# Autodesk Inventor assembly: Z Drive Assembly
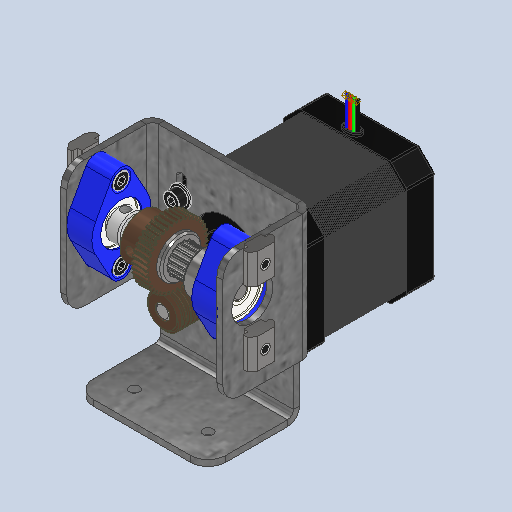
[picture p0: Inventor's stored thumbnail of the model, 512x512]
Saved by Autodesk Inventor 2022 (Build 260153000, 153)
## iProperties
Created: 2022-02-13
Part Number: Z Drive Assembly
Document SubType Name: Assembly
Designer: nicol
Author: nicol
## Documents named in this file (14)
- Y:\Projects\Bibble0\SubAsm\Z Drive Assembly.iam
- Y:\Projects\Bibble0\Sheet Metal\Z Drive Mount.ipt
- Y:\Projects\Bibble0\3D printed\Z Axis\Z Drive Bearing Holder.ipt
- Y:\Projects\Bibble0\Bearings\625 Bearing.ipt
- Y:\Projects\Bibble0\Hardware\5 x 50mm Shaft.ipt
- Y:\Projects\Bibble0\Hardware\GT2 Pulley 16T.ipt
- Y:\Projects\Bibble0\Hardware\METAL WORM GEAR_57545K624 v5.ipt
- Y:\Projects\Bibble0\Hardware\PLASTIC WORM GEAR_4037N115 v3.ipt
- Y:\Projects\Bibble0\Electronics\NEMA 17.ipt
- Y:\Projects\Bibble0\Hardware\M3 x 12 mm  SHCS.ipt
- Y:\Projects\Bibble0\Hardware\M3 T-Slot Nut.ipt
- Y:\Projects\Bibble0\Hardware\M3 x 6 mm SHCS.ipt
- Y:\Projects\Bibble0\Hardware\M3 Washer.ipt
- Y:\Projects\Bibble0\Hardware\5mm Collar.ipt
## Components (27 placed, 13 different names)
1. Z Drive Mount:1 — Insert:4, Insert:5, Insert:6, Mate:5, Insert:8, Insert:9, Insert:14, Insert:15, Insert:16, Insert:17, Angle:2, Angle:4, Insert:19, Insert:23, Insert:24, Insert:25
2. Z Drive Bearing Holder:1 — Insert:4, Insert:5, Insert:12, Insert:13
3. Z Drive Bearing Holder:2 — Insert:6, Insert:10, Insert:11
4. 625 Bearing:1 — Mate:4, Mate:6
5. 625 Bearing:2
6. 5 x 50mm Shaft:1 — Mate:4, Mate:7
7. GT2 Pulley 16T:1
8. METAL WORM GEAR_57545K624 v5:1 — Insert:7
9. PLASTIC WORM GEAR_4037N115 v3:1
10. NEMA 17:1 — Mate:5, Insert:7, Insert:8, Insert:9
11. M3 x 12 mm  SHCS:1 — Insert:10
12. M3 x 12 mm  SHCS:2 — Insert:12
13. M3 x 12 mm  SHCS:3 — Insert:11
14. M3 x 12 mm  SHCS:4 — Insert:13
15. M3 T-Slot Nut:1 — Insert:15, Angle:3, Angle:4
16. M3 T-Slot Nut:2 — Insert:17, Angle:1
17. M3 T-Slot Nut:3 — Insert:16, Angle:1, Angle:2
18. M3 T-Slot Nut:4 — Insert:14, Angle:3
19. M3 x 6 mm SHCS:1 — Insert:18
20. M3 Washer:1 — Insert:18, Insert:19
21. M3 x 6 mm SHCS:2
22. M3 Washer:2 — Insert:23
23. M3 x 6 mm SHCS:3
24. M3 Washer:3 — Insert:24
25. M3 x 6 mm SHCS:4
26. M3 Washer:4 — Insert:25
27. 5mm Collar:1 — Mate:6, Mate:7
## Relationships (37: Insert 25, Mate 7, Angle 4, Flush 1)
- [Insert]: Z Drive Bearing Holder:2 ↔ 625 Bearing:1
- [Insert]: Z Drive Bearing Holder:1 ↔ 625 Bearing:2
- [Mate]: 625 Bearing:2 ↔ 5 x 50mm Shaft:1
- [Flush]: 625 Bearing:2 ↔ 5 x 50mm Shaft:1
- [Insert]: GT2 Pulley 16T:1 ↔ PLASTIC WORM GEAR_4037N115 v3:1
- [Mate] (15 mm): Z Drive Bearing Holder:1 ↔ PLASTIC WORM GEAR_4037N115 v3:1
- [Mate]: 5 x 50mm Shaft:1 ↔ PLASTIC WORM GEAR_4037N115 v3:1
- Mate:4: 625 Bearing:1 ↔ 5 x 50mm Shaft:1
- Insert:4: Z Drive Mount:1 ↔ Z Drive Bearing Holder:1
- Insert:5: Z Drive Mount:1 ↔ Z Drive Bearing Holder:1
- Insert:6: Z Drive Mount:1 ↔ Z Drive Bearing Holder:2
- Mate:5: Z Drive Mount:1 ↔ NEMA 17:1
- Insert:7: METAL WORM GEAR_57545K624 v5:1 ↔ NEMA 17:1
- Insert:8: Z Drive Mount:1 ↔ NEMA 17:1
- Insert:9: Z Drive Mount:1 ↔ NEMA 17:1
- Insert:10: Z Drive Bearing Holder:2 ↔ M3 x 12 mm  SHCS:1
- Insert:11: Z Drive Bearing Holder:2 ↔ M3 x 12 mm  SHCS:3
- Insert:12: Z Drive Bearing Holder:1 ↔ M3 x 12 mm  SHCS:2
- Insert:13: Z Drive Bearing Holder:1 ↔ M3 x 12 mm  SHCS:4
- Insert:14: Z Drive Mount:1 ↔ M3 T-Slot Nut:4
- Insert:15: Z Drive Mount:1 ↔ M3 T-Slot Nut:1
- Insert:16: Z Drive Mount:1 ↔ M3 T-Slot Nut:3
- Insert:17: Z Drive Mount:1 ↔ M3 T-Slot Nut:2
- Angle:1 (0 deg): M3 T-Slot Nut:2 ↔ M3 T-Slot Nut:3
- Angle:2 (0 deg): Z Drive Mount:1 ↔ M3 T-Slot Nut:3
- Angle:3 (0 deg): M3 T-Slot Nut:1 ↔ M3 T-Slot Nut:4
- Angle:4 (0 deg): Z Drive Mount:1 ↔ M3 T-Slot Nut:1
- Insert:18: M3 x 6 mm SHCS:1 ↔ M3 Washer:1
- Insert:19: Z Drive Mount:1 ↔ M3 Washer:1
- [Insert]: M3 x 6 mm SHCS:2 ↔ M3 Washer:2
- [Insert]: M3 x 6 mm SHCS:3 ↔ M3 Washer:3
- [Insert]: M3 x 6 mm SHCS:4 ↔ M3 Washer:4
- Insert:23: Z Drive Mount:1 ↔ M3 Washer:2
- Insert:24: Z Drive Mount:1 ↔ M3 Washer:3
- Insert:25: Z Drive Mount:1 ↔ M3 Washer:4
- Mate:6: 625 Bearing:1 ↔ 5mm Collar:1
- Mate:7: 5 x 50mm Shaft:1 ↔ 5mm Collar:1
## Named parameters: d33_d31 = 0 mm, d34_d31 = 0 mm, d35_d31 = 0 mm
